# Autodesk Inventor assembly: ProbeHead V2 - Assembly
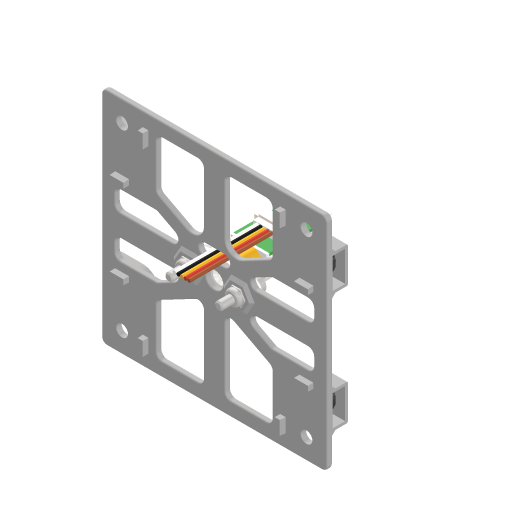
[picture p0: Inventor's stored thumbnail of the model, 512x512]
Saved by Autodesk Inventor 2023.2 (Build 272271000, 271)
## iProperties
Created: 2024-02-09
Part Number: ProbeHead V2 - Assembly
Document SubType Name: Assembly
Designer: Nils Bade
Author: Nils Bade
## Documents named in this file (7)
- C:\Users\nilsb\Documents\Inventor\Projektarbeit-Bade\RatRig_modified\ProbeHead\ProbeAntennas\BLTouch_Plate.iam
- C:\Users\nilsb\Documents\Inventor\Projektarbeit-Bade\Schrauben\Cap Head Screw M3x12 v2.ipt
- C:\Users\nilsb\Documents\Inventor\Projektarbeit-Bade\RatRig_modified\ProbeHead\BLTouch Sensor V3_1.ipt
- BL Touch Sensor.ipt
- C:\Users\nilsb\Documents\Inventor\Projektarbeit-Bade\RatRig_Standards\Hex Locking Nut - M3 v2.ipt
- C:\Users\nilsb\Documents\Inventor\Projektarbeit-Bade\RatRig_modified\ProbeHead\BLTouch-Leveling-Plate_V2.ipt
- C:\Users\nilsb\Documents\Inventor\Projektarbeit-Bade\Enclosure\Magnet-RatrigEnclosure.ipt
## Components (14 placed, 5 different names)
1. BLTouch-Leveling-Plate_V2:1 — Passend:84, Passend:85, Winkel:22, Winkel:23, Passend:88, Passend:89, Passend:100, Passend:101, Passend:102, Passend:103, Passend:104, Passend:105, Passend:106, Passend:107
2. BL Touch Sensor:1 — Passend:72, Passend:73, Passend:74, Passend:75
3. Hex Locking Nut - M3 v2:1 — Passend:87, Winkel:22, Passend:88
4. Hex Locking Nut - M3 v2:2 — Passend:86, Winkel:23, Passend:89
5. Cap Head Screw M3x12 v2:9 — Passend:72, Passend:75, Passend:85, Passend:86
6. Cap Head Screw M3x12 v2:10 — Passend:73, Passend:74, Passend:84, Passend:87
7. Magnet-RatrigEnclosure:1 — Passend:102, Passend:105
8. Magnet-RatrigEnclosure:2
9. Magnet-RatrigEnclosure:3
10. Magnet-RatrigEnclosure:4 — Passend:103, Passend:104
11. Magnet-RatrigEnclosure:5 — Passend:100, Passend:106
12. Magnet-RatrigEnclosure:6
13. Magnet-RatrigEnclosure:7 — Passend:101, Passend:107
14. Magnet-RatrigEnclosure:8
## Relationships (21: Mate 19, Angle 2)
- [Mate]: BLTouch-Leveling-Plate_V2:1 ↔ BL Touch Sensor:1
- Passend:72 [Mate]: BL Touch Sensor:1 ↔ Cap Head Screw M3x12 v2:9
- Passend:73 [Mate]: BL Touch Sensor:1 ↔ Cap Head Screw M3x12 v2:10
- Passend:74 [Mate]: BL Touch Sensor:1 ↔ Cap Head Screw M3x12 v2:10
- Passend:75 [Mate]: BL Touch Sensor:1 ↔ Cap Head Screw M3x12 v2:9
- Passend:84 [Mate]: BLTouch-Leveling-Plate_V2:1 ↔ Cap Head Screw M3x12 v2:10
- Passend:85 [Mate]: BLTouch-Leveling-Plate_V2:1 ↔ Cap Head Screw M3x12 v2:9
- Passend:86 [Mate]: Hex Locking Nut - M3 v2:2 ↔ Cap Head Screw M3x12 v2:9
- Passend:87 [Mate]: Hex Locking Nut - M3 v2:1 ↔ Cap Head Screw M3x12 v2:10
- Winkel:22 [Angle] (0 deg): BLTouch-Leveling-Plate_V2:1 ↔ Hex Locking Nut - M3 v2:1
- Winkel:23 [Angle] (0 deg): BLTouch-Leveling-Plate_V2:1 ↔ Hex Locking Nut - M3 v2:2
- Passend:88 [Mate]: BLTouch-Leveling-Plate_V2:1 ↔ Hex Locking Nut - M3 v2:1
- Passend:89 [Mate]: BLTouch-Leveling-Plate_V2:1 ↔ Hex Locking Nut - M3 v2:2
- Passend:100 [Mate]: BLTouch-Leveling-Plate_V2:1 ↔ Magnet-RatrigEnclosure:5
- Passend:101 [Mate]: BLTouch-Leveling-Plate_V2:1 ↔ Magnet-RatrigEnclosure:7
- Passend:102 [Mate]: BLTouch-Leveling-Plate_V2:1 ↔ Magnet-RatrigEnclosure:1
- Passend:103 [Mate]: BLTouch-Leveling-Plate_V2:1 ↔ Magnet-RatrigEnclosure:4
- Passend:104 [Mate]: BLTouch-Leveling-Plate_V2:1 ↔ Magnet-RatrigEnclosure:4
- Passend:105 [Mate]: BLTouch-Leveling-Plate_V2:1 ↔ Magnet-RatrigEnclosure:1
- Passend:106 [Mate]: BLTouch-Leveling-Plate_V2:1 ↔ Magnet-RatrigEnclosure:5
- Passend:107 [Mate]: BLTouch-Leveling-Plate_V2:1 ↔ Magnet-RatrigEnclosure:7
